# Autodesk Inventor assembly: pixhawk+carrello
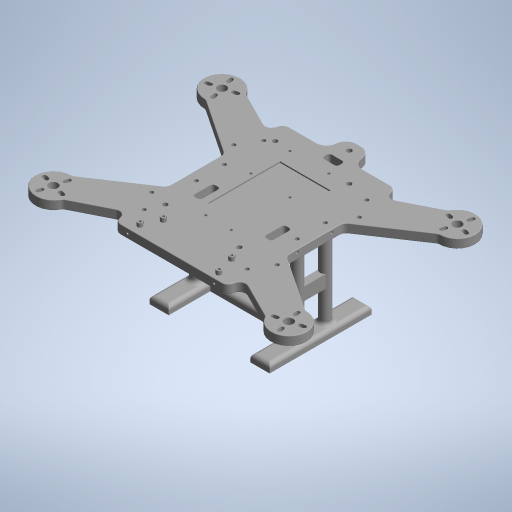
[picture p0: Inventor's stored thumbnail of the model, 512x512]
Saved by Autodesk Inventor 2023.2 (Build 272271030, 271C)
## iProperties
Part Number: pixhawk+carrello
Document SubType Name: Assembly
Designer: matti
Author: matti
## Documents named in this file (3)
- C:\Users\matti\OneDrive\Documenti\Università\Magistrale\Design methods for industrial engineering\DroneProject\pixhawk+carrello.iam
- C:\Users\matti\OneDrive\Documenti\Università\Magistrale\Design methods for industrial engineering\DroneProject\airframe_pixhawk_v2.ipt
- C:\Users\matti\OneDrive\Documenti\Università\Magistrale\Design methods for industrial engineering\DroneProject\carrello.ipt
## Components (2 placed, 2 different names)
1. airframe_pixhawk_v2:1 — Insert:1
2. carrello:1 — Insert:1
## Relationships (1: Insert 1)
- Insert:1: airframe_pixhawk_v2:1 ↔ carrello:1
